# Autodesk Inventor assembly: matrix_V2
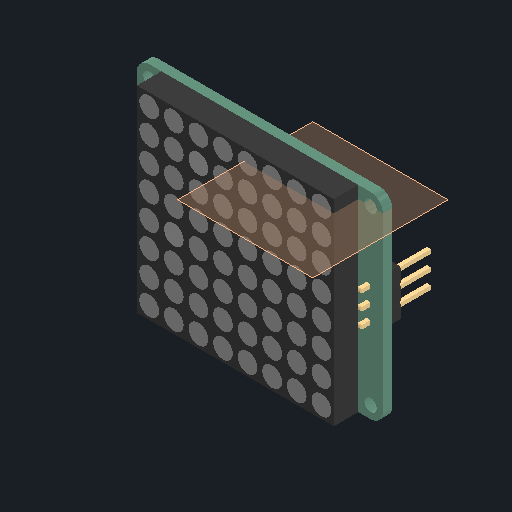
[picture p0: Inventor's stored thumbnail of the model, 512x512]
Saved by Autodesk Inventor 2025.2 (Build 292293000, 293)
## iProperties
Created: 2025-11-14
Part Number: matrix_V2
Document SubType Name: Assembly
Designer: micyg
Author: micyg
## Documents named in this file (3)
- D:\Projects\VirtualPets\VirtualBlob\Mechanical\matrix\matrix_V2.iam
- D:\Projects\VirtualPets\VirtualBlob\Mechanical\boards\MatrixBoard_0_0_0\MatrixBoard.iam
- D:\Projects\VirtualPets\VirtualBlob\Mechanical\matrix\matrixDiffuser.ipt
## Components (2 placed, 2 different names)
1. MatrixBoard:1 [sub-assembly] — Mate:1, Flush:1, Flush:2
2. matrixDiffuser:1 — Mate:1, Flush:1, Flush:2
## Relationships (3: Flush 2, Mate 1)
- Mate:1: MatrixBoard:1 ↔ matrixDiffuser:1
- Flush:1: MatrixBoard:1 ↔ matrixDiffuser:1
- Flush:2 (4 mm): MatrixBoard:1 ↔ matrixDiffuser:1
